# Autodesk Inventor assembly: Card Cage
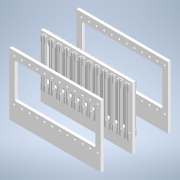
[picture p0: Inventor's stored thumbnail of the model, 180x180]
Saved by Autodesk Inventor 2021 (Build 250183000, 183)
## iProperties
Created: 2022-07-24
Part Number: Card Cage
Document SubType Name: Assembly
Designer: erics
Author: erics
## Documents named in this file (3)
- D:\Users\erics\Documents\16B\Mechanical\Card Cage.iam
- D:\Users\erics\Documents\16B\Mechanical\Center Wall.ipt
- D:\Users\erics\Documents\16B\Mechanical\CCA Rail.ipt
## Components (27 placed, 2 different names)
1. Center Wall:1 — Insert:1, Insert:2, Insert:3, Insert:4, Mate:1, Mate:2, Mate:3, Flush:1, Flush:2, Flush:3, Flush:4, Flush:5, Flush:6
2. Center Wall:2 — Flush:1, Flush:2, Flush:3
3. Center Wall:3 — Flush:4, Flush:5, Flush:6
4. CCA Rail:2 — Insert:3, Insert:4
5. CCA Rail:1 — Insert:1, Insert:2
6. CCA Rail:3
7. CCA Rail:4
8. CCA Rail:5
9. CCA Rail:6
10. CCA Rail:7
11. CCA Rail:8
12. CCA Rail:9
13. CCA Rail:10
14. CCA Rail:11
15. CCA Rail:12
16. CCA Rail:13
17. CCA Rail:14
18. CCA Rail:15
19. CCA Rail:16
20. CCA Rail:17
21. CCA Rail:18
22. CCA Rail:19
23. CCA Rail:20
24. CCA Rail:21
25. CCA Rail:22
26. CCA Rail:23
27. CCA Rail:24
## Component patterns: (12 elements, first: CCA Rail:2 + CCA Rail:1)
## Relationships (13: Flush 6, Insert 4, Mate 3)
- Insert:1: Center Wall:1 ↔ CCA Rail:1
- Insert:2: Center Wall:1 ↔ CCA Rail:1
- Insert:3: Center Wall:1 ↔ CCA Rail:2
- Insert:4: Center Wall:1 ↔ CCA Rail:2
- Mate:1: Center Wall:1
- Mate:2: Center Wall:1
- Mate:3: Center Wall:1
- Flush:1: Center Wall:1 ↔ Center Wall:2
- Flush:2: Center Wall:1 ↔ Center Wall:2
- Flush:3 (73.66 mm): Center Wall:1 ↔ Center Wall:2
- Flush:4: Center Wall:1 ↔ Center Wall:3
- Flush:5: Center Wall:1 ↔ Center Wall:3
- Flush:6 (83.82 mm): Center Wall:1 ↔ Center Wall:3
